# Autodesk Inventor assembly: Baugruppe1
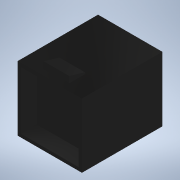
[picture p0: Inventor's stored thumbnail of the model, 180x180]
Saved by Autodesk Inventor 2020 (Build 240168000, 168)
## iProperties
Created: 2021-05-12
Part Number: Baugruppe1
Document SubType Name: Assembly
Designer: Julian Uhl
Author: Julian Uhl
## Documents named in this file (5)
- C:\Users\Julian Uhl\Desktop\Eier-Inventor\Baugruppe1.iam
- C:\Users\Julian Uhl\Desktop\Eier-Inventor\Bauteil1.ipt
- C:\Users\Julian Uhl\Desktop\Eier-Inventor\Gitter.ipt
- C:\Users\Julian Uhl\Desktop\Eier-Inventor\Ei.ipt
- C:\Users\Julian Uhl\Desktop\Eier-Inventor\Ei_groß.ipt
## Components (6 placed, 4 different names)
1. Bauteil1:1 — Passend:1, Passend:2, Passend:3
2. Gitter:1 — Passend:1, Passend:2, Passend:3
3. Ei:3
4. Ei:4
5. Ei_groß:1
6. Ei_groß:2
## Relationships (3: Mate 3)
- Passend:1 [Mate]: Bauteil1:1 ↔ Gitter:1
- Passend:2 [Mate]: Bauteil1:1 ↔ Gitter:1
- Passend:3 [Mate]: Bauteil1:1 ↔ Gitter:1
